# Autodesk Inventor assembly: Proto
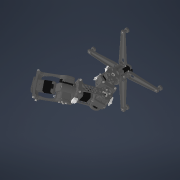
[picture p0: Inventor's stored thumbnail of the model, 180x180]
Saved by Autodesk Inventor 2022 (Build 260153070, 153G)
## iProperties
Created: 2021-11-24
Part Number: Proto
Document SubType Name: Assembly
Designer: Teo
Title: Predstavitev sklopa
Author: Teo
## Documents named in this file (6)
- D:\Zaključna\Roka\Priloge\STL_files\Assemblies\Proto.iam
- D:\Zaključna\Roka\Priloge\IPT_files\Assemblies\base_link.iam
- D:\Zaključna\Roka\Priloge\IPT_files\Assemblies\shoulder_link.iam
- D:\Zaključna\Roka\Priloge\IPT_files\Assemblies\short_link.iam
- D:\Zaključna\Roka\Priloge\IPT_files\Assemblies\long_link.iam
- D:\Zaključna\Roka\Priloge\IPT_files\Assemblies\plate_link.iam
## Components (7 placed, 5 different names)
1. base_link:1 [sub-assembly] — Rotational:1
2. shoulder_link:1 [sub-assembly] — Rotational:1, Rotational:2
3. short_link:1 [sub-assembly] — Rotational:2, Rotational:3
4. long_link:1 [sub-assembly] — Rotational:3, Rotational:4
5. shoulder_link:2 [sub-assembly] — Rotational:4, Rotational:5
6. long_link:2 [sub-assembly] — Rotational:5, Rotational:6
7. plate_link:1 [sub-assembly] — Rotational:6
## Relationships (6: RevoluteJoint 6)
- Rotational:1 [RevoluteJoint]: base_link:1 ↔ shoulder_link:1
- Rotational:2 [RevoluteJoint]: shoulder_link:1 ↔ short_link:1
- Rotational:3 [RevoluteJoint]: short_link:1 ↔ long_link:1
- Rotational:4 [RevoluteJoint]: long_link:1 ↔ shoulder_link:2
- Rotational:5 [RevoluteJoint]: shoulder_link:2 ↔ long_link:2
- Rotational:6 [RevoluteJoint]: long_link:2 ↔ plate_link:1
